# Autodesk Inventor assembly: OBG-Oberbau
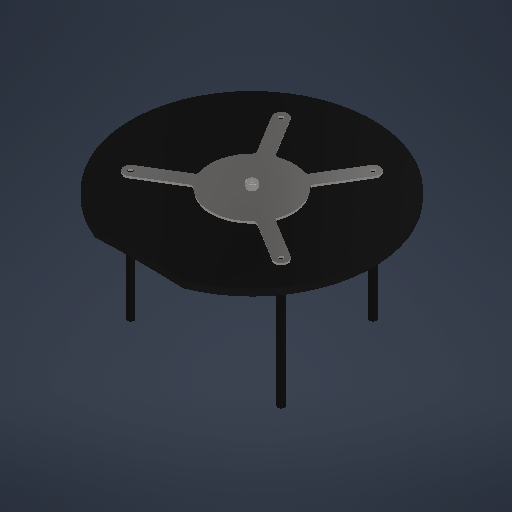
[picture p0: Inventor's stored thumbnail of the model, 512x512]
Saved by Autodesk Inventor 2025.2 (Build 292293000, 293)
## iProperties
Created: 2025-03-28
Part Number: OBG-Oberbau
Document SubType Name: Assembly
Designer: Faabs
Author: Faabs
## Documents named in this file (6)
- C:\Users\Faabs\Desktop\TeamFaabs-CAD v2023\OBG\OBG-Oberbau.iam
- C:\Users\Faabs\Desktop\TeamFaabs-CAD v2023\OBG\Spiegelhalterung.ipt
- C:\Users\Faabs\Desktop\TeamFaabs-CAD v2023\OBG\Spiegel.ipt
- C:\Users\Faabs\Desktop\TeamFaabs-CAD v2023\OBG\Spiegelabdeckung\Spiegelabdeckung\Spiegelabdeckung.ipt
- C:\Users\Faabs\Desktop\TeamFaabs-CAD v2023\OBG\Abstandshalter.ipt
- C:\Users\Faabs\Desktop\TeamFaabs-CAD v2023\Verbindungselemente\DIN 912\DIN 912 - M4 x 0,7 x 6 x 4,25.ipt
## Components (8 placed, 5 different names)
1. Spiegelhalterung:1 — Passend:1, Passend:2, Passend:3, Passend:4, Passend:5, Einfügen:1, Passend:6, Passend:7, Passend:8
2. Spiegel:1 — Passend:4, Passend:5
3. Abstandshalter:1 — Passend:10, Passend:14
4. Abstandshalter:2 — Passend:12, Passend:16
5. Abstandshalter:3 — Passend:9, Passend:13
6. Abstandshalter:4 — Passend:11, Passend:15
7. Spiegelabdeckung:1 — Passend:6, Passend:7, Passend:8, Passend:9, Passend:10, Passend:11, Passend:12, Passend:13, Passend:14, Passend:15, Passend:16
8. DIN 912 - ersetzt durch DIN EN ISO 4762 M4 x 6:1 — Einfügen:1
## Relationships (17: Mate 16, Insert 1)
- Passend:1 [Mate]: Spiegelhalterung:1
- Passend:2 [Mate]: Spiegelhalterung:1
- Passend:3 [Mate]: Spiegelhalterung:1
- Passend:4 [Mate]: Spiegelhalterung:1 ↔ Spiegel:1
- Passend:5 [Mate]: Spiegelhalterung:1 ↔ Spiegel:1
- Einfügen:1 [Insert]: Spiegelhalterung:1 ↔ DIN 912 - ersetzt durch DIN EN ISO 4762 M4 x 6:1
- Passend:6 [Mate]: Spiegelhalterung:1 ↔ Spiegelabdeckung:1
- Passend:7 [Mate]: Spiegelhalterung:1 ↔ Spiegelabdeckung:1
- Passend:8 [Mate]: Spiegelhalterung:1 ↔ Spiegelabdeckung:1
- Passend:9 [Mate]: Abstandshalter:3 ↔ Spiegelabdeckung:1
- Passend:10 [Mate]: Abstandshalter:1 ↔ Spiegelabdeckung:1
- Passend:11 [Mate]: Abstandshalter:4 ↔ Spiegelabdeckung:1
- Passend:12 [Mate]: Abstandshalter:2 ↔ Spiegelabdeckung:1
- Passend:13 [Mate]: Abstandshalter:3 ↔ Spiegelabdeckung:1
- Passend:14 [Mate]: Abstandshalter:1 ↔ Spiegelabdeckung:1
- Passend:15 [Mate]: Abstandshalter:4 ↔ Spiegelabdeckung:1
- Passend:16 [Mate]: Abstandshalter:2 ↔ Spiegelabdeckung:1
